# Autodesk Inventor assembly: Ensamblaje lanzador
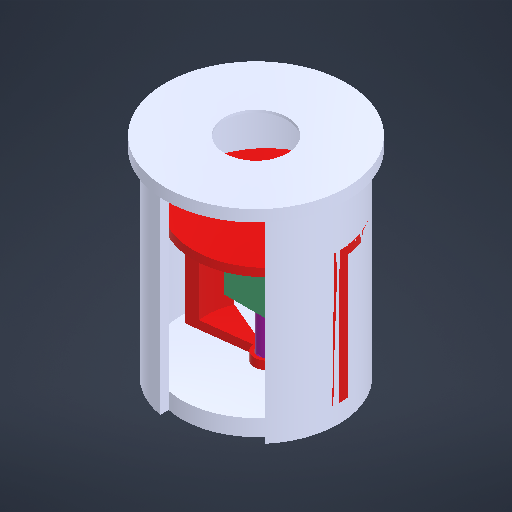
[picture p0: Inventor's stored thumbnail of the model, 512x512]
Saved by Autodesk Inventor 2026.2 (Build 302298010, 298A)
## iProperties
Created: 1601-01-04
Part Number: Ensamblaje lanzador
Document SubType Name: Assembly
Designer: trini
Sending System: SOLIDWORKS 2016
Last Saved Date: 2025-09-02
last saved by: tgreco
Author: trini
## Documents named in this file (7)
- C:\Users\trini\OneDrive - ITBA\ITBA\Tesis\Solid lanzador\Solid lanzador\Ensamblaje lanzador.iam
- C:\Users\trini\OneDrive - ITBA\ITBA\Tesis\Solid lanzador\Solid lanzador\Ensamblaje lanzador\Ensamblaje lanzador\Lanzador cilindrico.ipt
- C:\Users\trini\OneDrive - ITBA\ITBA\Tesis\Solid lanzador\Solid lanzador\Ensamblaje lanzador\Ensamblaje lanzador\Lanzador cilindrico p2.ipt
- C:\Users\trini\OneDrive - ITBA\ITBA\Tesis\Solid lanzador\Solid lanzador\Ensamblaje lanzador\Ensamblaje lanzador\modelo solenoide.ipt
- C:\Users\trini\OneDrive - ITBA\ITBA\Tesis\Solid lanzador\Solid lanzador\Ensamblaje lanzador\Ensamblaje lanzador\palito.ipt
- C:\Users\trini\OneDrive - ITBA\ITBA\Tesis\Solid lanzador\Solid lanzador\Ensamblaje lanzador\Ensamblaje lanzador\tapa lanzador.ipt
- C:\Users\trini\OneDrive - ITBA\ITBA\Tesis\Solid lanzador\Solid lanzador\Ensamblaje lanzador\Ensamblaje lanzador\tapa pelota.ipt
## Components (6 placed, 6 different names)
1. Lanzador cilindrico-1 — Rigid:1, Insert:3, Insert:4
2. Lanzador cilindrico p2-1 — Insert:2
3. modelo solenoide-1 — Insert:1, Rigid:1
4. palito-1 — Insert:1, Insert:2
5. tapa lanzador-1 — Insert:3
6. tapa pelota-1 — Insert:4
## Relationships (5: Insert 4, WeldJoint 1)
- Insert:1: modelo solenoide-1 ↔ palito-1
- Rigid:1 [WeldJoint]: Lanzador cilindrico-1 ↔ modelo solenoide-1
- Insert:2: Lanzador cilindrico p2-1 ↔ palito-1
- Insert:3: Lanzador cilindrico-1 ↔ tapa lanzador-1
- Insert:4: Lanzador cilindrico-1 ↔ tapa pelota-1
